# Autodesk Inventor assembly: REV-11-1271
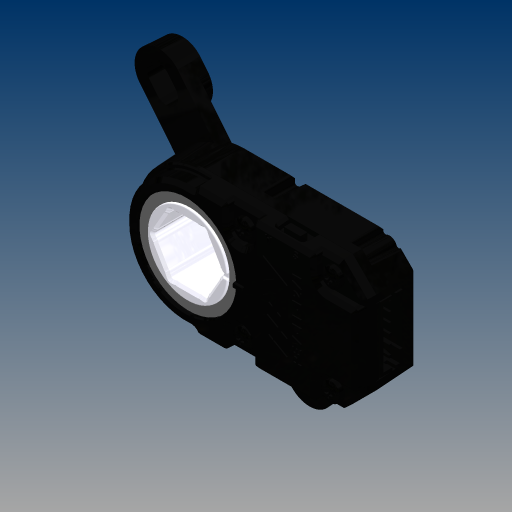
[picture p0: Inventor's stored thumbnail of the model, 512x512]
Saved by Autodesk Inventor 2024.3 (Build 283343000, 343)
## iProperties
Created: 2019-08-05
Part Number: REV-11-1271
Description: STEP AP203
Document SubType Name: Assembly
Designer: Kenji
Title: REV-11-1271.STEP
Revision Number: ANY
Sending System: SolidWorks 2018
Preprocessor: SwSTEP 2.0
## Documents named in this file (11)
- C:\Users\Kenji\Documents\GitHub\1622-2024-Summer-CAD-A-Thon\Intake\REV-11-1271(ThroughBoreEncoder).iam
- C:\Users\Kenji\Downloads\REV-11-1271\REV-11-1271\REV-11-1271-1.ipt
- C:\Users\Kenji\Downloads\REV-11-1271\REV-11-1271\REV-11-1271-4.ipt
- C:\Users\Kenji\Downloads\REV-11-1271\REV-11-1271\REV-11-1271-0.ipt
- C:\Users\Kenji\Downloads\REV-11-1271\REV-11-1271\6703-ZZ Bearing.ipt
- C:\Users\Kenji\Downloads\REV-11-1271\REV-11-1271\128-2Z Bearing_7804K145.ipt
- C:\Users\Kenji\Downloads\REV-11-1271\REV-11-1271\REV-11-1271-5.ipt
- C:\Users\Kenji\Downloads\REV-11-1271\REV-11-1271\S6B-PH-K-S.ipt
- C:\Users\Kenji\Downloads\REV-11-1271\REV-11-1271\cross recessed thread forming screws gb_GB_CROSS_SCREWS_TYPE138 M2X8X7.2-N.ipt
- C:\Users\Kenji\Downloads\REV-11-1271\REV-11-1271\REV-11-1271-3 Alt.ipt
- C:\Users\Kenji\Downloads\REV-11-1271\REV-11-1271\REV-11-1271-2 ALT.ipt
## Components (14 placed, 14 different names)
1. REV-11-1271-1_1
2. REV-11-1271-4_2
3. REV-11-1271-0_3
4. 6703-ZZ Bearing_4
5. 128-2Z Bearing_7804K145_5
6. REV-11-1271-5_6
7. S6B-PH-K-S_7
8. cross recessed thread forming screws gb_GB_CROSS_SCREWS_TYPE138 M2X8X7.2-N_8
9. cross recessed thread forming screws gb_GB_CROSS_SCREWS_TYPE138 M2X8X7.2-N_9
10. cross recessed thread forming screws gb_GB_CROSS_SCREWS_TYPE138 M2X8X7.2-N_10
11. cross recessed thread forming screws gb_GB_CROSS_SCREWS_TYPE138 M2X8X7.2-N_11
12. REV-11-1271-3 Alt_12
13. 6703-ZZ Bearing_13
14. REV-11-1271-2 ALT_14
## Named parameters: Finish1_Area = 163.831, Finish2_Area = 163.831, Finish3_Area = 12.278, Finish4_Area = 3.76991
note: some values were not read from the file. Shown as the stored number, unit unknown: "Finish1_Area", "Finish2_Area", "Finish3_Area", "Finish4_Area".
